# Autodesk Inventor assembly: tempAsm
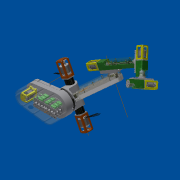
[picture p0: Inventor's stored thumbnail of the model, 180x180]
Saved by Autodesk Inventor 2018 (Build 220112000, 112)
## iProperties
Created: 2020-03-07
Part Number: tempAsm
Document SubType Name: Assembly
Designer: Bunny320
Author: Bunny320
## Documents named in this file (7)
- C:\Users\Bunny320\Desktop\sechs\4-CAD\tempAsm.iam
- C:\Users\Bunny320\Desktop\sechs\4-CAD\10-J1.iam
- C:\Users\Bunny320\Desktop\sechs\4-CAD\20-J2.iam
- C:\Users\Bunny320\Desktop\sechs\4-CAD\30-J3.iam
- C:\Users\Bunny320\Desktop\sechs\4-CAD\40-J4.iam
- C:\Users\Bunny320\Desktop\sechs\4-CAD\50-J5.iam
- C:\Users\Bunny320\Desktop\sechs\4-CAD\60-J6(ref J5).iam
## Components (6 placed, 6 different names)
1. 10-J1:1 [sub-assembly] — Flush:1, Flush:2, Flush:3, Mate:1, Mate:2, Mate:3, Mate:4, Mate:5, Mate:6
2. 20-J2:1 [sub-assembly] — Mate:1, Mate:2, Mate:3, Flush:4
3. 30-J3:1 [sub-assembly] — Mate:4, Mate:5, Mate:6, Flush:4, Mate:51, Mate:52
4. 40-J4:1 [sub-assembly] — Mate:51, Mate:52, Mate:53, Mate:54
5. 50-J5:1 [sub-assembly] — Mate:53, Mate:54, Mate:55, Mate:56
6. 60-J6(ref J5):1 [sub-assembly] — Mate:55, Mate:56
## Relationships (16: Mate 12, Flush 4)
- Flush:1: 10-J1:1
- Flush:2: 10-J1:1
- Flush:3: 10-J1:1
- Mate:1: 10-J1:1 ↔ 20-J2:1
- Mate:2: 10-J1:1 ↔ 20-J2:1
- Mate:3: 10-J1:1 ↔ 20-J2:1
- Mate:4: 10-J1:1 ↔ 30-J3:1
- Mate:5: 10-J1:1 ↔ 30-J3:1
- Mate:6: 10-J1:1 ↔ 30-J3:1
- Flush:4: 20-J2:1 ↔ 30-J3:1
- Mate:51: 30-J3:1 ↔ 40-J4:1
- Mate:52: 30-J3:1 ↔ 40-J4:1
- Mate:53: 40-J4:1 ↔ 50-J5:1
- Mate:54: 40-J4:1 ↔ 50-J5:1
- Mate:55: 50-J5:1 ↔ 60-J6(ref J5):1
- Mate:56: 50-J5:1 ↔ 60-J6(ref J5):1
